# Autodesk Inventor assembly: obudowa_elektroniki
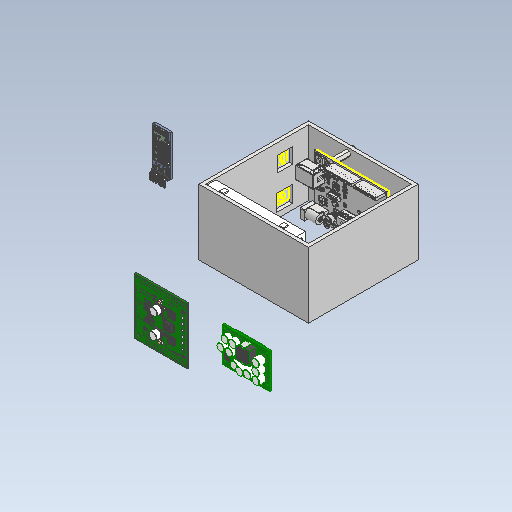
[picture p0: Inventor's stored thumbnail of the model, 512x512]
Saved by Autodesk Inventor 2020 (Build 240168000, 168)
## iProperties
Created: 2020-08-10
Part Number: obudowa_elektroniki
Document SubType Name: Assembly
Designer: Hesekiel
Author: Hesekiel
## Documents named in this file (10)
- C:\Users\Hesekiel\Desktop\Equatorial-Mount-MUM\Mechanika\Obudowa elektroniki\CAD\obudowa_elektroniki.iam
- C:\Users\Hesekiel\Desktop\Equatorial-Mount-MUM\Mechanika\Obudowa elektroniki\CAD\Sterownik silnika - Dual TB9051FTG.ipt
- C:\Users\Hesekiel\Desktop\Equatorial-Mount-MUM\Mechanika\Obudowa elektroniki\CAD\Konwerter step-down - D24V150FX.ipt
- C:\Users\Hesekiel\Desktop\Equatorial-Mount-MUM\Mechanika\Obudowa elektroniki\CAD\obudowa.ipt
- C:\Users\Hesekiel\Desktop\Equatorial-Mount-MUM\Mechanika\Obudowa elektroniki\CAD\arduino-uno-r3-1.snapshot.3\arduino uno.iam
- C:\Users\Hesekiel\Desktop\Equatorial-Mount-MUM\Mechanika\Obudowa elektroniki\CAD\HC_05 Blue Tooth Module.ipt
- C:\Users\Hesekiel\Desktop\Equatorial-Mount-MUM\Mechanika\Obudowa elektroniki\CAD\HalfBreadboard.ipt
- C:\Users\Hesekiel\Desktop\Equatorial-Mount-MUM\Mechanika\Obudowa elektroniki\CAD\Standoff_M3_14mm.ipt
- C:\Users\Hesekiel\Desktop\Equatorial-Mount-MUM\Mechanika\Obudowa elektroniki\CAD\DIN 934 - M3 x 0.5.ipt
- C:\Users\Hesekiel\Desktop\Equatorial-Mount-MUM\Mechanika\Obudowa elektroniki\CAD\DIN 912 - M3 x 0.5 x 6 x 4.75.ipt
## Components (18 placed, 9 different names)
1. Sterownik silnika - Dual TB9051FTG:1
2. Konwerter step-down - D24V150FX:1
3. obudowa:1 — Mate:1, Mate:2, Mate:3, Mate:4, Flush:1, Mate:5, Mate:6, Mate:7, Mate:8, Mate:9, Mate:10, Mate:11, Mate:12, Mate:13, Mate:15, Mate:16, Mate:17
4. arduino uno:1 [sub-assembly] — Mate:1, Mate:2, Mate:21, Mate:22, Mate:23, Mate:24, Mate:25, Mate:26, Mate:27, Mate:28, Mate:29
5. HC_05 Blue Tooth Module:1
6. HalfBreadboard:1 — Mate:3, Mate:4, Flush:1
7. Standoff_M3_14mm:1 — Mate:5, Mate:6, Mate:14, Mate:21
8. Standoff_M3_14mm:2 — Mate:9, Mate:10, Mate:19
9. Standoff_M3_14mm:3 — Mate:11, Mate:12, Mate:18
10. Standoff_M3_14mm:4 — Mate:7, Mate:8, Mate:20
11. DIN 934 - replaced by DIN EN 24032/28673/28674 M3:1 — Mate:16, Mate:19
12. DIN 934 - replaced by DIN EN 24032/28673/28674 M3:2 — Mate:13, Mate:14
13. DIN 934 - replaced by DIN EN 24032/28673/28674 M3:3 — Mate:15, Mate:20
14. DIN 934 - replaced by DIN EN 24032/28673/28674 M3:4 — Mate:17, Mate:18
15. DIN 912 - replaced by DIN EN ISO 4762 M3 x 6:1 — Mate:22, Mate:23
16. DIN 912 - replaced by DIN EN ISO 4762 M3 x 6:2 — Mate:24, Mate:25
17. DIN 912 - replaced by DIN EN ISO 4762 M3 x 6:3 — Mate:26, Mate:27
18. DIN 912 - replaced by DIN EN ISO 4762 M3 x 6:4 — Mate:28, Mate:29
## Relationships (30: Mate 29, Flush 1)
- Mate:1: obudowa:1 ↔ arduino uno:1
- Mate:2: obudowa:1 ↔ arduino uno:1
- Mate:3: obudowa:1 ↔ HalfBreadboard:1
- Mate:4: obudowa:1 ↔ HalfBreadboard:1
- Flush:1: obudowa:1 ↔ HalfBreadboard:1
- Mate:5: obudowa:1 ↔ Standoff_M3_14mm:1
- Mate:6: obudowa:1 ↔ Standoff_M3_14mm:1
- Mate:7: obudowa:1 ↔ Standoff_M3_14mm:4
- Mate:8: obudowa:1 ↔ Standoff_M3_14mm:4
- Mate:9: obudowa:1 ↔ Standoff_M3_14mm:2
- Mate:10: obudowa:1 ↔ Standoff_M3_14mm:2
- Mate:11: obudowa:1 ↔ Standoff_M3_14mm:3
- Mate:12: obudowa:1 ↔ Standoff_M3_14mm:3
- Mate:13: obudowa:1 ↔ DIN 934 - replaced by DIN EN 24032/28673/28674 M3:2
- Mate:14: Standoff_M3_14mm:1 ↔ DIN 934 - replaced by DIN EN 24032/28673/28674 M3:2
- Mate:15: obudowa:1 ↔ DIN 934 - replaced by DIN EN 24032/28673/28674 M3:3
- Mate:16: obudowa:1 ↔ DIN 934 - replaced by DIN EN 24032/28673/28674 M3:1
- Mate:17: obudowa:1 ↔ DIN 934 - replaced by DIN EN 24032/28673/28674 M3:4
- Mate:18: Standoff_M3_14mm:3 ↔ DIN 934 - replaced by DIN EN 24032/28673/28674 M3:4
- Mate:19: Standoff_M3_14mm:2 ↔ DIN 934 - replaced by DIN EN 24032/28673/28674 M3:1
- Mate:20: Standoff_M3_14mm:4 ↔ DIN 934 - replaced by DIN EN 24032/28673/28674 M3:3
- Mate:21: arduino uno:1 ↔ Standoff_M3_14mm:1
- Mate:22: arduino uno:1 ↔ DIN 912 - replaced by DIN EN ISO 4762 M3 x 6:1
- Mate:23: arduino uno:1 ↔ DIN 912 - replaced by DIN EN ISO 4762 M3 x 6:1
- Mate:24: arduino uno:1 ↔ DIN 912 - replaced by DIN EN ISO 4762 M3 x 6:2
- Mate:25: arduino uno:1 ↔ DIN 912 - replaced by DIN EN ISO 4762 M3 x 6:2
- Mate:26: arduino uno:1 ↔ DIN 912 - replaced by DIN EN ISO 4762 M3 x 6:3
- Mate:27: arduino uno:1 ↔ DIN 912 - replaced by DIN EN ISO 4762 M3 x 6:3
- Mate:28: arduino uno:1 ↔ DIN 912 - replaced by DIN EN ISO 4762 M3 x 6:4
- Mate:29: arduino uno:1 ↔ DIN 912 - replaced by DIN EN ISO 4762 M3 x 6:4
